# Autodesk Inventor assembly: triangle_brace
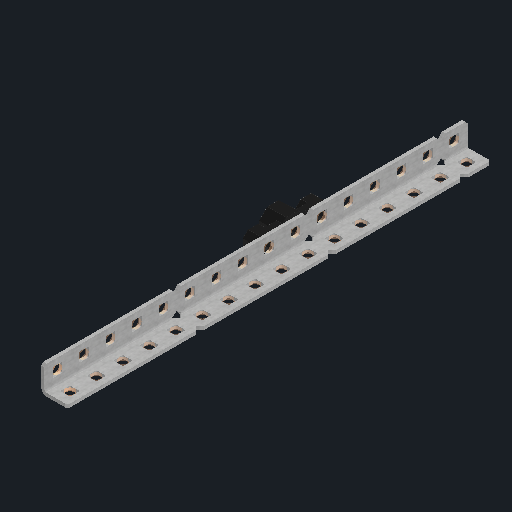
[picture p0: Inventor's stored thumbnail of the model, 512x512]
Saved by Autodesk Inventor 2025 (Build 290162000, 162)
## iProperties
Created: 2024-10-13
Part Number: triangle_brace
Document SubType Name: Assembly
Designer: Averey Ku
Author: Averey Ku
## Documents named in this file (3)
- D:\vex_robotics_high_stakes\hardware\cad\bots\high_stakes_v2\tower\structure\triangle_brace.iam
- D:\vex_robotics_high_stakes\hardware\cad\robpros_cad_lib\Structure\Angle\Aluminum 1x1\Alu Angle 1x1x16.ipt
- D:\vex_robotics_high_stakes\hardware\cad\robpros_cad_lib\Motion\Shaft HS\HS Bearing Flat.ipt
## Components (2 placed, 2 different names)
1. Alu Angle 1x1x16:1 — Mate:2, Angle:1, Mate:3, Flush:1
2. HS Bearing Flat:1
## Relationships (6: Mate 3, Insert 1, Angle 1, Flush 1)
- [Insert]: Alu Angle 1x1x16:1 ↔ HS Bearing Flat:1
- [Mate]: Alu Angle 1x1x16:1 ↔ HS Bearing Flat:1
- Mate:2 (6.35 mm): Alu Angle 1x1x16:1
- Angle:1 (0 deg): Alu Angle 1x1x16:1
- Mate:3: Alu Angle 1x1x16:1
- Flush:1: Alu Angle 1x1x16:1
